# Autodesk Inventor assembly: ASSY,ROBOT,2026
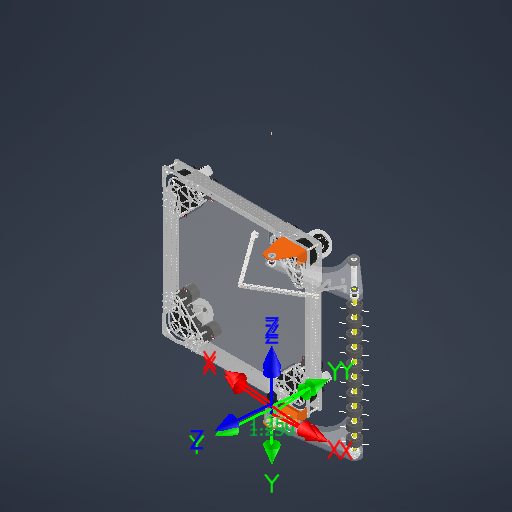
[picture p0: Inventor's stored thumbnail of the model, 512x512]
Saved by Autodesk Inventor 2026.1 (Build 301233020, 233B)
## iProperties
Created: 2026-01-24
Part Number: ASSY,ROBOT,2026
Document SubType Name: Assembly
Designer: Jthib
Mass: 24729.3 g
Surface Area: 49621.3 cm^2
Volume: 29693.7 cm^3
Density: 0.832814 g/cm^3
Author: Jthib
## Documents named in this file (4)
- C:\Users\joejp\OneDrive\Documents\GitHub\2026-Robot-Mechanical\ASSY,ROBOT,2026.iam
- C:\Users\joejp\OneDrive\Documents\GitHub\2026-Robot-Mechanical\Chassis\CHASSIS.iam
- C:\Users\joejp\OneDrive\Documents\GitHub\2026-Robot-Mechanical\Chassis\Bumpers.ipt
- E:\Inventor\Rebuilt\Workspaces\Workspace\InputAssembly.iam
## Components (3 placed, 3 different names)
1. CHASSIS:1 [sub-assembly] — Flush:1, Flush:2, Flush:3, Flush:4, Mate:1, Mate:2, Mate:3, Position Intake ForeAff, Postion Intake Side2Side, Mate:4
2. Bumpers:1 — Flush:4, Mate:1, Mate:2
3. InputAssembly:1 [sub-assembly] — Mate:3, Position Intake ForeAff, Postion Intake Side2Side, Mate:4
## Relationships (10: Flush 6, Mate 4)
- Flush:1 (-349.25 mm): CHASSIS:1
- Flush:2 (349.25 mm): CHASSIS:1
- Flush:3: CHASSIS:1
- Flush:4 (-12.7 mm): CHASSIS:1 ↔ Bumpers:1
- Mate:1: CHASSIS:1 ↔ Bumpers:1
- Mate:2: CHASSIS:1 ↔ Bumpers:1
- Mate:3: CHASSIS:1 ↔ InputAssembly:1
- Position Intake ForeAff [Flush] (3.175 mm): CHASSIS:1 ↔ InputAssembly:1
- Postion Intake Side2Side [Flush] (1.5875 mm): CHASSIS:1 ↔ InputAssembly:1
- Mate:4: CHASSIS:1 ↔ InputAssembly:1
